# Autodesk Inventor assembly: Assembly1
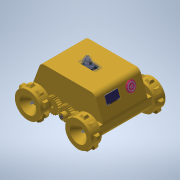
[picture p0: Inventor's stored thumbnail of the model, 180x180]
Saved by Autodesk Inventor 2020 (Build 240168000, 168)
## iProperties
Created: 2020-01-27
Part Number: Assembly1
Document SubType Name: Assembly
Designer: blep
Author: blep
## Documents named in this file (21)
- C:\Users\blep\Desktop\ScanBot\3d-model\Assembly1.iam
- C:\Users\blep\Desktop\ScanBot\3d-model\Tower Pro MG90S Micro servo\Tower Pro MG90S Micro servo.iam
- C:\Users\blep\Documents\Inventor\Content Center Files\R2020\pl-PL\AS 1427(08)\AS 1427 - M4 x 16(6) I.ipt
- C:\Users\blep\Desktop\ScanBot\3d-model\wheel.ipt
- C:\Users\blep\Desktop\ScanBot\3d-model\wheel_MIR.ipt
- C:\Users\blep\Desktop\ScanBot\3d-model\wheel_FRONT.ipt
- C:\Users\blep\Desktop\ScanBot\3d-model\wheel_FRONT_MIR.ipt
- C:\Users\blep\Desktop\ScanBot\3d-model\MG996R servo\MG_996R.iam
- C:\Users\blep\Desktop\ScanBot\3d-model\led on off push button\16mm-LED-Power-Button.iam
- C:\Users\blep\Desktop\ScanBot\3d-model\base-v2.ipt
- C:\Users\blep\Desktop\ScanBot\3d-model\small-gear-v2.ipt
- C:\Users\blep\Desktop\ScanBot\3d-model\small-gear-v2_MIR.ipt
- C:\Users\blep\Desktop\ScanBot\3d-model\EC11 encoder - long\EC11_Rotary_Encoder_Switched.ipt
- C:\Users\blep\Desktop\ScanBot\3d-model\small-gear-v2_CPY.ipt
- C:\Users\blep\Desktop\ScanBot\3d-model\18650 battery\18650.ipt
- C:\Users\blep\Desktop\ScanBot\3d-model\small-gear-v2_CPY_MIR.ipt
- C:\Users\blep\Desktop\ScanBot\3d-model\lm2596 buck converter\LM2596 DC-DC StepDown Converter v1.ipt
- C:\Users\blep\Desktop\ScanBot\3d-model\motherboard.ipt
- C:\Users\blep\Desktop\ScanBot\3d-model\1306 OLED 128x64 I2C 0.96 inch\OSSD-128x64.ipt
- C:\Users\blep\Desktop\ScanBot\3d-model\cover-new.ipt
- C:\Users\blep\Documents\Inventor\Content Center Files\R2020\pl-PL\AS 1112 (2)\AS 1112 - M4  Typ 5.ipt
## Components (32 placed, 20 different names)
1. base-v2:1 — Zestawiające:6, Zestawiające:9, Zestawiające:10, Obrotowe:1, Obrotowe:6, Obrotowe:2, Obrotowe:3, Równoległe:16, Równoległe:17, Zestawiające:11, Zestawiające:12, Zestawiające:13, Sztywne:1, Sztywne:2, Sztywne:3, Sztywne:4, Zestawiające:14, Styczny:3, Styczny:4, Styczny:5, Styczny:9, Sztywne:5, Sztywne:6, Kątowe:1, Kątowe:16, Kątowe:17, Kątowe:18, Równoległe:21, Równoległe:22, Sztywne:16
2. small-gear-v2:1 — Obrotowe:7
3. small-gear-v2_MIR:1 — Obrotowe:8
4. small-gear-v2_CPY:1 — Obrotowe:9
5. small-gear-v2_CPY_MIR:1 — Obrotowe:10
6. motherboard:1 — Zestawiające:15, Równoległe:21, Równoległe:22
7. cover-new:1 — Sztywne:7, Zestawiające:16, Zestawiające:17, Zestawiające:18, Sztywne:9, Sztywne:10, Sztywne:13, Sztywne:14, Sztywne:15, Sztywne:16
8. AS 1112 (2) - Metryczny M4  Typ 5:1 — Sztywne:10
9. AS 1112 (2) - Metryczny M4  Typ 5:2 — Sztywne:15
10. AS 1112 (2) - Metryczny M4  Typ 5:3 — Sztywne:14
11. AS 1112 (2) - Metryczny M4  Typ 5:4 — Sztywne:9
12. wheel:1 — Obrotowe:6
13. wheel_MIR:1 — Obrotowe:1
14. wheel_FRONT:1 — Obrotowe:3
15. wheel_FRONT_MIR:1 — Obrotowe:2
16. AS 1427 Z - Metryczny M4 x 16:8 — Sztywne:4
17. AS 1427 Z - Metryczny M4 x 16:9 — Sztywne:1
18. AS 1427 Z - Metryczny M4 x 16:10 — Sztywne:3
19. AS 1427 Z - Metryczny M4 x 16:13 — Sztywne:2
20. 16mm-LED-Power-Button:1 [sub-assembly] — Sztywne:7
21. MG_996R:1 [sub-assembly] — Równoległe:15, Równoległe:17, Zestawiające:12, Obrotowe:8
22. MG_996R:2 [sub-assembly] — Równoległe:15, Równoległe:16, Obrotowe:7, Zestawiające:11, Zestawiające:13, Zestawiające:15
23. 18650:1 — Styczny:1, Równoległe:18, Zestawiające:14, Styczny:3
24. 18650:2 — Styczny:1, Równoległe:18, Styczny:4, Równoległe:20, Styczny:7, Styczny:8
25. 18650:3 — Styczny:2, Równoległe:19, Styczny:5, Równoległe:20, Styczny:7, Styczny:9
26. 18650:4 — Styczny:2, Równoległe:19, Styczny:8
27. EC11_Rotary_Encoder_Switched:1 — Sztywne:6, Obrotowe:10
28. EC11_Rotary_Encoder_Switched:2 — Sztywne:5, Obrotowe:9
29. LM2596 DC-DC StepDown Converter v1:1 — Kątowe:16, Kątowe:17
30. LM2596 DC-DC StepDown Converter v1:2 — Kątowe:1, Kątowe:18
31. OSSD-128x64:1 — Zestawiające:16, Zestawiające:17, Zestawiające:18
32. Tower Pro MG90S Micro servo:3 [sub-assembly] — Sztywne:13
## Relationships (52: WeldJoint 13, Mate 11, RevoluteJoint 8, Flush 8, Tangent 8, Angle 4)
- Zestawiające:6 [Mate]: base-v2:1
- Zestawiające:9 [Mate]: base-v2:1
- Zestawiające:10 [Mate]: base-v2:1
- Obrotowe:1 [RevoluteJoint] (-0.5 mm): base-v2:1 ↔ wheel_MIR:1
- Obrotowe:6 [RevoluteJoint] (0.5 mm): base-v2:1 ↔ wheel:1
- Obrotowe:2 [RevoluteJoint] (-0.5 mm): base-v2:1 ↔ wheel_FRONT_MIR:1
- Obrotowe:3 [RevoluteJoint] (0.5 mm): base-v2:1 ↔ wheel_FRONT:1
- Równoległe:15 [Flush]: MG_996R:1 ↔ MG_996R:2
- Równoległe:16 [Flush] (0.5 mm): base-v2:1 ↔ MG_996R:2
- Równoległe:17 [Flush] (0.5 mm): base-v2:1 ↔ MG_996R:1
- Obrotowe:7 [RevoluteJoint] (-0.2 mm): small-gear-v2:1 ↔ MG_996R:2
- Zestawiające:11 [Mate]: base-v2:1 ↔ MG_996R:2
- Zestawiające:12 [Mate]: base-v2:1 ↔ MG_996R:1
- Zestawiające:13 [Mate] (4.7 mm): base-v2:1 ↔ MG_996R:2
- Obrotowe:8 [RevoluteJoint] (-0.2 mm): small-gear-v2_MIR:1 ↔ MG_996R:1
- Sztywne:1 [WeldJoint]: base-v2:1 ↔ AS 1427 Z - Metryczny M4 x 16:9
- Sztywne:2 [WeldJoint]: base-v2:1 ↔ AS 1427 Z - Metryczny M4 x 16:13
- Sztywne:3 [WeldJoint]: base-v2:1 ↔ AS 1427 Z - Metryczny M4 x 16:10
- Sztywne:4 [WeldJoint]: base-v2:1 ↔ AS 1427 Z - Metryczny M4 x 16:8
- Styczny:1 [Tangent]: 18650:1 ↔ 18650:2
- Styczny:2 [Tangent]: 18650:3 ↔ 18650:4
- Równoległe:18 [Flush]: 18650:1 ↔ 18650:2
- Równoległe:19 [Flush]: 18650:3 ↔ 18650:4
- Zestawiające:14 [Mate] (7.5 mm): base-v2:1 ↔ 18650:1
- Styczny:3 [Tangent]: base-v2:1 ↔ 18650:1
- Styczny:4 [Tangent]: base-v2:1 ↔ 18650:2
- Styczny:5 [Tangent]: base-v2:1 ↔ 18650:3
- Równoległe:20 [Flush]: 18650:2 ↔ 18650:3
- Styczny:7 [Tangent]: 18650:2 ↔ 18650:3
- Styczny:8 [Tangent]: 18650:2 ↔ 18650:4
- Styczny:9 [Tangent] (0.5 mm): base-v2:1 ↔ 18650:3
- Sztywne:5 [WeldJoint]: base-v2:1 ↔ EC11_Rotary_Encoder_Switched:2
- Obrotowe:9 [RevoluteJoint] (16.7 mm): small-gear-v2_CPY:1 ↔ EC11_Rotary_Encoder_Switched:2
- Sztywne:6 [WeldJoint]: base-v2:1 ↔ EC11_Rotary_Encoder_Switched:1
- Obrotowe:10 [RevoluteJoint] (-16.7 mm): small-gear-v2_CPY_MIR:1 ↔ EC11_Rotary_Encoder_Switched:1
- Kątowe:1 [Angle] (0 deg): base-v2:1 ↔ LM2596 DC-DC StepDown Converter v1:2
- Kątowe:16 [Angle] (0 deg): base-v2:1 ↔ LM2596 DC-DC StepDown Converter v1:1
- Kątowe:17 [Angle] (0 deg): base-v2:1 ↔ LM2596 DC-DC StepDown Converter v1:1
- Kątowe:18 [Angle] (0 deg): base-v2:1 ↔ LM2596 DC-DC StepDown Converter v1:2
- Zestawiające:15 [Mate]: motherboard:1 ↔ MG_996R:2
- Równoległe:21 [Flush] (10 mm): base-v2:1 ↔ motherboard:1
- Równoległe:22 [Flush] (10 mm): base-v2:1 ↔ motherboard:1
- Sztywne:7 [WeldJoint]: cover-new:1 ↔ 16mm-LED-Power-Button:1
- Zestawiające:16 [Mate]: cover-new:1 ↔ OSSD-128x64:1
- Zestawiające:17 [Mate] (1 mm): cover-new:1 ↔ OSSD-128x64:1
- Zestawiające:18 [Mate] (1 mm): cover-new:1 ↔ OSSD-128x64:1
- Sztywne:9 [WeldJoint]: cover-new:1 ↔ AS 1112 (2) - Metryczny M4  Typ 5:4
- Sztywne:10 [WeldJoint]: cover-new:1 ↔ AS 1112 (2) - Metryczny M4  Typ 5:1
- Sztywne:13 [WeldJoint]: cover-new:1 ↔ Tower Pro MG90S Micro servo:3
- Sztywne:14 [WeldJoint]: cover-new:1 ↔ AS 1112 (2) - Metryczny M4  Typ 5:3
- Sztywne:15 [WeldJoint]: cover-new:1 ↔ AS 1112 (2) - Metryczny M4  Typ 5:2
- Sztywne:16 [WeldJoint]: base-v2:1 ↔ cover-new:1
